# Autodesk Inventor assembly: Logger
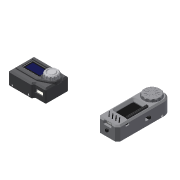
[picture p0: Inventor's stored thumbnail of the model, 180x180]
Saved by Autodesk Inventor 2020 (Build 240168000, 168)
## iProperties
Created: 2022-10-11
Part Number: Logger
Document SubType Name: Assembly
Designer: uch10113
Author: uch10113
## Documents named in this file (15)
- \\hc.hucoag.net\hcdfs0001\hc0001\CH_Huba_E\Technologie\ND\Zeichungen\T2\Logger\Logger.iam
- \\hc.hucoag.net\hcdfs0001\hc0001\CH_Huba_E\Technologie\ND\Zeichungen\T2\Logger\C3.ipt
- \\hc.hucoag.net\hcdfs0001\hc0001\CH_Huba_E\Technologie\ND\Zeichungen\T2\Logger\OLED 128x64.ipt
- \\hc.hucoag.net\hcdfs0001\hc0001\CH_Huba_E\Technologie\ND\Zeichungen\T2\Logger\encoder.ipt
- \\hc.hucoag.net\hcdfs0001\hc0001\CH_Huba_E\Technologie\ND\Zeichungen\T2\Logger\Battery.ipt
- \\hc.hucoag.net\hcdfs0001\hc0001\CH_Huba_E\Technologie\ND\Zeichungen\T2\Logger\Knoob.ipt
- \\hc.hucoag.net\hcdfs0001\hc0001\CH_Huba_E\Technologie\ND\Zeichungen\T2\Logger\HousingTop.ipt
- \\hc.hucoag.net\hcdfs0001\hc0001\CH_Huba_E\Technologie\ND\Zeichungen\T2\Logger\Boden.ipt
- \\hc.hucoag.net\hcdfs0001\hc0001\CH_Huba_E\Technologie\ND\Zeichungen\T2\Logger\Adapter.ipt
- \\hc.hucoag.net\hcdfs0001\hc0001\CH_Huba_E\Technologie\ND\Zeichungen\Einlogger\T-Display.iam
- \\hc.hucoag.net\hcdfs0001\hc0001\CH_Huba_E\Technologie\ND\Zeichungen\T2\Logger\LoggerTdisplay\Displaydeckel.ipt
- \\hc.hucoag.net\hcdfs0001\hc0001\CH_Huba_E\Technologie\ND\Zeichungen\T2\Logger\LoggerTdisplay\Knoonb.ipt
- \\hc.hucoag.net\hcdfs0001\hc0001\CH_Huba_E\Technologie\ND\Zeichungen\T2\Logger\LoggerTdisplay\Niederhalter.ipt
- \\hc.hucoag.net\hcdfs0001\hc0001\CH_Huba_E\Technologie\ND\Zeichungen\T2\Logger\LoggerTdisplay\boden.ipt
- \\hc.hucoag.net\hcdfs0001\hc0001\CH_Huba_E\Technologie\ND\Zeichungen\T2\Logger\LoggerTdisplay\SS12F15.iam
## Components (15 placed, 14 different names)
1. C3:1 — Winkel:1, Passend:1, Fluchtend:1, Fluchtend:2, Passend:2, Fluchtend:5, Fluchtend:7
2. OLED 128x64:1 — Winkel:1, Passend:1, Fluchtend:1, Fluchtend:2, Fluchtend:4, Fluchtend:8
3. encoder:1 — Passend:3, Fluchtend:3, Passend:4, Passend:5, Passend:6
4. Battery:1 — Passend:2, Passend:3, Fluchtend:3, Passend:5, Fluchtend:5
5. Knoob:1 — Passend:4, Passend:6
6. HousingTop:1 — Fluchtend:4, Fluchtend:6
7. Boden:1 — Fluchtend:6
8. Adapter:1 — Fluchtend:7, Fluchtend:8
9. T-Display:1 [sub-assembly] — Passend:7, Passend:8, Passend:9, Passend:15
10. Displaydeckel:1 — Passend:7, Passend:8, Passend:9, Passend:10, Passend:11, Passend:12, Fluchtend:9, Fluchtend:10, Fluchtend:11, Passend:13, Passend:14
11. Knoonb:1 — Passend:10, Passend:11, Passend:12
12. Niederhalter:1 — Fluchtend:9, Fluchtend:12, Fluchtend:13
13. boden:1 — Fluchtend:10, Fluchtend:11
14. SS12F15:1 [sub-assembly] — Passend:13
15. SS12F15:2 [sub-assembly] — Passend:14, Passend:15, Fluchtend:12, Fluchtend:13
## Relationships (29: Mate 15, Flush 13, Angle 1)
- Winkel:1 [Angle] (0 deg): C3:1 ↔ OLED 128x64:1
- Passend:1 [Mate] (2 mm): C3:1 ↔ OLED 128x64:1
- Fluchtend:1 [Flush]: C3:1 ↔ OLED 128x64:1
- Fluchtend:2 [Flush] (3.05 mm): C3:1 ↔ OLED 128x64:1
- Passend:2 [Mate] (1 mm): C3:1 ↔ Battery:1
- Passend:3 [Mate]: encoder:1 ↔ Battery:1
- Fluchtend:3 [Flush]: encoder:1 ↔ Battery:1
- Passend:4 [Mate]: encoder:1 ↔ Knoob:1
- Passend:5 [Mate] (0.5 mm): encoder:1 ↔ Battery:1
- Passend:6 [Mate] (3 mm): encoder:1 ↔ Knoob:1
- Fluchtend:4 [Flush]: OLED 128x64:1 ↔ HousingTop:1
- Fluchtend:5 [Flush]: C3:1 ↔ Battery:1
- Fluchtend:6 [Flush]: HousingTop:1 ↔ Boden:1
- Fluchtend:7 [Flush]: C3:1 ↔ Adapter:1
- Fluchtend:8 [Flush]: OLED 128x64:1 ↔ Adapter:1
- Passend:7 [Mate]: T-Display:1 ↔ Displaydeckel:1
- Passend:8 [Mate] (0.3 mm): T-Display:1 ↔ Displaydeckel:1
- Passend:9 [Mate] (0.3 mm): T-Display:1 ↔ Displaydeckel:1
- Passend:10 [Mate] (1.5 mm): Displaydeckel:1 ↔ Knoonb:1
- Passend:11 [Mate]: Displaydeckel:1 ↔ Knoonb:1
- Passend:12 [Mate] (1.5 mm): Displaydeckel:1 ↔ Knoonb:1
- Fluchtend:9 [Flush]: Displaydeckel:1 ↔ Niederhalter:1
- Fluchtend:10 [Flush]: Displaydeckel:1 ↔ boden:1
- Fluchtend:11 [Flush]: Displaydeckel:1 ↔ boden:1
- Passend:13 [Mate] (1 mm): Displaydeckel:1 ↔ SS12F15:1
- Passend:14 [Mate] (2 mm): Displaydeckel:1 ↔ SS12F15:2
- Passend:15 [Mate] (2 mm): T-Display:1 ↔ SS12F15:2
- Fluchtend:12 [Flush] (8.5 mm): Niederhalter:1 ↔ SS12F15:2
- Fluchtend:13 [Flush]: Niederhalter:1 ↔ SS12F15:2
